# Autodesk Inventor assembly: Prototy-1
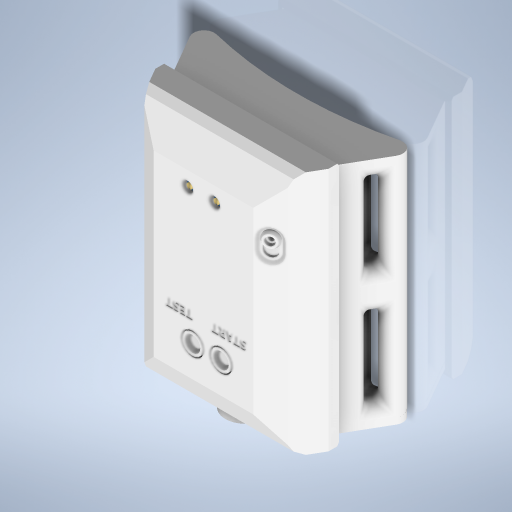
[picture p0: Inventor's stored thumbnail of the model, 512x512]
Saved by Autodesk Inventor 2024.3 (Build 283343000, 343)
## iProperties
Created: 2025-01-22
Part Number: Prototy-1
Document SubType Name: Assembly
Designer: ASUS TUF
Author: ASUS TUF
## Documents named in this file (14)
- C:\Users\ASUS TUF\Documents\Inventor\ParkinsonDetection\Prototy-1.iam
- C:\Users\ASUS TUF\Documents\Inventor\ParkinsonDetection\PCB-V1.ipt
- C:\Users\ASUS TUF\Documents\Inventor\ParkinsonDetection\3296W\3296W\3296W.ipt
- C:\Users\ASUS TUF\Documents\Inventor\ParkinsonDetection\LiPo-650mAh.ipt
- C:\Users\ASUS TUF\Documents\Inventor\ParkinsonDetection\LP112527-3.7V650mAh\LP112527-3.7V650mAh\LP112527-3.7V650mAh.ipt
- C:\Users\ASUS TUF\Documents\Inventor\ParkinsonDetection\Switch.ipt
- C:\Users\ASUS TUF\Documents\Inventor\ParkinsonDetection\TACTILE SWITCH\TACTILE SWITCH\TACTILE SWITCH.ipt
- C:\Users\ASUS TUF\Documents\Inventor\ParkinsonDetection\Holder-PCB.ipt
- C:\Users\ASUS TUF\Documents\Inventor\ParkinsonDetection\Case-Bottom.ipt
- C:\Users\ASUS TUF\Documents\Inventor\ParkinsonDetection\Socket.ipt
- C:\Users\ASUS TUF\Documents\Inventor\ParkinsonDetection\Pin.ipt
- C:\Users\ASUS TUF\Documents\Inventor\ParkinsonDetection\Buzzer.ipt
- C:\Users\ASUS TUF\Documents\Inventor\ParkinsonDetection\XIAO-nRF52840 v15\XIAO-nRF52840 v15\XIAO-nRF52840 v15.iam
- C:\Users\ASUS TUF\Documents\Inventor\ParkinsonDetection\Pin_MIR.ipt
## Components (16 placed, 13 different names)
1. Case-Bottom:1 — Flush:14, Mate:16, Tangent:1, Flush:23, Tangent:2, Flush:24, Flush:25, Flush:26, Flush:28, Flush:29
2. LiPo-650mAh:1 — Flush:7, Angle:1, Mate:13, Mate:14, Symmetry:1, Tangent:1
3. LP112527-3.7V650mAh:1 — Mate:9, Angle:2, Mate:13, Mate:14, Mate:15, Flush:13, Symmetry:1, Tangent:3
4. PCB-V1:1 — Mate:1, Mate:2, Flush:1, Flush:2, Flush:3, Flush:4, Flush:5, Mate:4, Mate:5, Mate:6, Flush:6, Flush:7, Mate:9, Flush:9, Mate:8, Flush:12, Angle:1, Angle:2, Mate:10, Mate:11, Mate:12, Mate:15, Flush:13, Flush:14, Flush:15, Mate:17, Mate:19, Flush:29, Mate:24, Mate:25
5. Holder-PCB:1 — Mate:10, Mate:11, Mate:12, Flush:26
6. 3296W:1 — Mate:1, Mate:3, Flush:5
7. 3296W:2 — Mate:2, Mate:3, Flush:4, Mate:4, Mate:18, Mate:20
8. Switch:1 — Mate:5, Mate:6, Flush:6, Flush:16
9. TACTILE SWITCH:1 — Mate:7, Flush:10, Flush:11
10. TACTILE SWITCH:2 — Mate:7, Flush:9, Flush:10, Flush:11, Mate:8, Flush:12
11. Socket:1 — Flush:15, Mate:17, Mate:18
12. Socket:2 — Mate:19, Mate:20, Flush:16
13. Pin:1 — Flush:22, Flush:23, Tangent:2, Flush:24, Flush:25
14. Buzzer:1 — Flush:27, Tangent:3, Flush:28
15. XIAO-nRF52840 v15:1 [sub-assembly] — Mate:24, Mate:25
16. Pin_MIR:1 — Flush:30
## Relationships (57: Mate 25, Flush 25, Angle 3, Tangent 3, Symmetry 1)
- Mate:1: PCB-V1:1 ↔ 3296W:1
- Mate:2: PCB-V1:1 ↔ 3296W:2
- Flush:1: PCB-V1:1
- Flush:2: PCB-V1:1
- Flush:3: PCB-V1:1
- Mate:3 (6 mm): 3296W:1 ↔ 3296W:2
- Flush:4 (2 mm): PCB-V1:1 ↔ 3296W:2
- Flush:5 (2 mm): PCB-V1:1 ↔ 3296W:1
- Mate:4 (17 mm): PCB-V1:1 ↔ 3296W:2
- Mate:5: PCB-V1:1 ↔ Switch:1
- Mate:6 (-5.5 mm): PCB-V1:1 ↔ Switch:1
- Flush:6 (4 mm): PCB-V1:1 ↔ Switch:1
- Flush:7: LiPo-650mAh:1 ↔ PCB-V1:1
- Mate:9: LP112527-3.7V650mAh:1 ↔ PCB-V1:1
- Mate:7 (5 mm): TACTILE SWITCH:1 ↔ TACTILE SWITCH:2
- Flush:9 (12.2 mm): PCB-V1:1 ↔ TACTILE SWITCH:2
- Flush:10: TACTILE SWITCH:1 ↔ TACTILE SWITCH:2
- Flush:11: TACTILE SWITCH:1 ↔ TACTILE SWITCH:2
- Mate:8 (-6 mm): PCB-V1:1 ↔ TACTILE SWITCH:2
- Flush:12 (11.5 mm): PCB-V1:1 ↔ TACTILE SWITCH:2
- Angle:1 (180 deg): LiPo-650mAh:1 ↔ PCB-V1:1
- Angle:2 (180 deg): LP112527-3.7V650mAh:1 ↔ PCB-V1:1
- Mate:10: PCB-V1:1 ↔ Holder-PCB:1
- Mate:11: PCB-V1:1 ↔ Holder-PCB:1
- Mate:12 (0.2 mm): PCB-V1:1 ↔ Holder-PCB:1
- Mate:13 (-3.5 mm): LiPo-650mAh:1 ↔ LP112527-3.7V650mAh:1
- Mate:14 (15 mm): LiPo-650mAh:1 ↔ LP112527-3.7V650mAh:1
- Mate:15 (10 mm): LP112527-3.7V650mAh:1 ↔ PCB-V1:1
- Flush:13 (-5 mm): LP112527-3.7V650mAh:1 ↔ PCB-V1:1
- Flush:14: Case-Bottom:1 ↔ PCB-V1:1
- Symmetry:1: LiPo-650mAh:1 ↔ LP112527-3.7V650mAh:1
- Mate:16: Case-Bottom:1
- Flush:15 (4 mm): PCB-V1:1 ↔ Socket:1
- Mate:17 (-7.5 mm): PCB-V1:1 ↔ Socket:1
- Mate:18 (6 mm): 3296W:2 ↔ Socket:1
- Mate:19 (-7.5 mm): PCB-V1:1 ↔ Socket:2
- Mate:20 (12.3 mm): 3296W:2 ↔ Socket:2
- Flush:16 (-7 mm): Switch:1 ↔ Socket:2
- Tangent:1: Case-Bottom:1 ↔ LiPo-650mAh:1
- Flush:21 (-172.9993 mm)
- Mate:21
- Mate:22
- Mate:23
- Angle:3 (7.64 deg)
- Flush:22: Pin:1
- Flush:23: Case-Bottom:1 ↔ Pin:1
- Tangent:2 (-1 mm): Case-Bottom:1 ↔ Pin:1
- Flush:24: Case-Bottom:1 ↔ Pin:1
- Flush:25: Case-Bottom:1 ↔ Pin:1
- Flush:26 (0.2 mm): Case-Bottom:1 ↔ Holder-PCB:1
- Flush:27: Buzzer:1
- Tangent:3 (2 mm): LP112527-3.7V650mAh:1 ↔ Buzzer:1
- Flush:28 (-3 mm): Case-Bottom:1 ↔ Buzzer:1
- Flush:29: Case-Bottom:1 ↔ PCB-V1:1
- Mate:24: PCB-V1:1 ↔ XIAO-nRF52840 v15:1
- Mate:25 (-17 mm): PCB-V1:1 ↔ XIAO-nRF52840 v15:1
- Flush:30: Pin_MIR:1
